# Autodesk Inventor assembly: boil-2
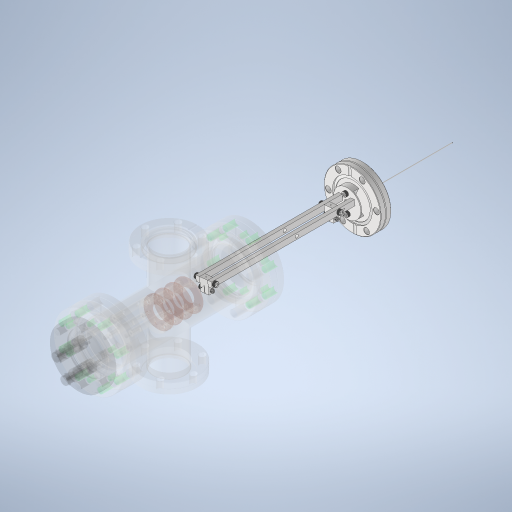
[picture p0: Inventor's stored thumbnail of the model, 512x512]
Saved by Autodesk Inventor 2024 (Build 280153000, 153)
## iProperties
Created: 2023-04-29
Part Number: boil-2
Document SubType Name: Assembly
Designer: Fujitsu
Author: Fujitsu
## Documents named in this file (10)
- C:\Users\Fujitsu\Raad\BaTag\dff275x000\boil-2.iam
- C:\Users\Fujitsu\Raad\BaTag\dff275x000\dff275x000-drilled-2.ipt
- C:\Users\Fujitsu\Raad\BaTag\capillary-2.ipt
- C:\Users\Fujitsu\Raad\BaTag\detector_chamber3\detector_chamber3.iam
- C:\Users\Fujitsu\Raad\BaTag\tab4.ipt
- C:\Users\Fujitsu\Raad\BaTag\rod(6-32).ipt
- C:\Users\Fujitsu\Raad\BaTag\clamp(6-32)-th.ipt
- C:\Users\Fujitsu\Raad\BaTag\ssVScrew(6-32).ipt
- C:\Users\Fujitsu\Raad\BaTag\tee.iam
- C:\Users\Fujitsu\Raad\BaTag\zwj.ipt
## Components (20 placed, 9 different names)
1. dff275x000-drilled-2:1 — Mate:1, Angle:1, Angle:2, Angle:3, Mate:4, Mate:5, Angle:4, Angle:5, Mate:17
2. capillary-2:1 — Mate:1, Angle:1, Mate:2, Mate:3, Mate:6, Mate:11, Mate:15, Mate:16, Mate:18
3. detector_chamber3:1 [sub-assembly] — Angle:2, Mate:2, Mate:3, Mate:20
4. tab4:1 — Angle:3, Mate:4, Mate:5, Mate:6, Mate:7, Mate:8, Mate:9, Mate:10, Insert:1, Insert:2, Insert:3, Insert:4
5. rod(6-32):1 — Mate:9, Mate:10, Angle:4, Mate:12, Mate:13, Mate:14, Insert:5, Insert:8
6. rod(6-32):2 — Mate:7, Mate:8, Angle:5, Insert:9, Insert:10
7. clamp(6-32)-th:1 — Mate:14, Mate:15, Insert:6
8. clamp(6-32)-th:2 — Mate:11, Mate:12, Mate:13, Insert:7
9. ssVScrew(6-32):1 — Insert:8
10. ssVScrew(6-32):2 — Insert:7
11. ssVScrew(6-32):3 — Insert:6
12. ssVScrew(6-32):4 — Insert:5
13. ssVScrew(6-32):5 — Insert:3
14. ssVScrew(6-32):6 — Insert:4
15. ssVScrew(6-32):7 — Insert:2
16. ssVScrew(6-32):8 — Insert:1
17. ssVScrew(6-32):9 — Insert:10
18. ssVScrew(6-32):10 — Insert:9
19. tee:1 [sub-assembly] — Mate:16, Mate:17, Mate:19
20. zwj:1 — Mate:18, Mate:19, Mate:20
## Relationships (35: Mate 20, Insert 10, Angle 5)
- Mate:1: dff275x000-drilled-2:1 ↔ capillary-2:1
- Angle:1 (90 deg): dff275x000-drilled-2:1 ↔ capillary-2:1
- Angle:2 (180 deg): dff275x000-drilled-2:1 ↔ detector_chamber3:1
- Mate:2: capillary-2:1 ↔ detector_chamber3:1
- Mate:3 (15 mm): capillary-2:1 ↔ detector_chamber3:1
- Angle:3 (180 deg): dff275x000-drilled-2:1 ↔ tab4:1
- Mate:4: dff275x000-drilled-2:1 ↔ tab4:1
- Mate:5: dff275x000-drilled-2:1 ↔ tab4:1
- Mate:6: capillary-2:1 ↔ tab4:1
- Mate:7: tab4:1 ↔ rod(6-32):2
- Mate:8: tab4:1 ↔ rod(6-32):2
- Mate:9: tab4:1 ↔ rod(6-32):1
- Mate:10: tab4:1 ↔ rod(6-32):1
- Angle:4 (0 deg): dff275x000-drilled-2:1 ↔ rod(6-32):1
- Angle:5 (0 deg): dff275x000-drilled-2:1 ↔ rod(6-32):2
- Mate:11: capillary-2:1 ↔ clamp(6-32)-th:2
- Mate:12: rod(6-32):1 ↔ clamp(6-32)-th:2
- Mate:13: rod(6-32):1 ↔ clamp(6-32)-th:2
- Mate:14: rod(6-32):1 ↔ clamp(6-32)-th:1
- Mate:15: capillary-2:1 ↔ clamp(6-32)-th:1
- Insert:1: tab4:1 ↔ ssVScrew(6-32):8
- Insert:2: tab4:1 ↔ ssVScrew(6-32):7
- Insert:3: tab4:1 ↔ ssVScrew(6-32):5
- Insert:4: tab4:1 ↔ ssVScrew(6-32):6
- Insert:5: rod(6-32):1 ↔ ssVScrew(6-32):4
- Insert:6: clamp(6-32)-th:1 ↔ ssVScrew(6-32):3
- Insert:7: clamp(6-32)-th:2 ↔ ssVScrew(6-32):2
- Insert:8: rod(6-32):1 ↔ ssVScrew(6-32):1
- Insert:9: rod(6-32):2 ↔ ssVScrew(6-32):10
- Insert:10: rod(6-32):2 ↔ ssVScrew(6-32):9
- Mate:16: capillary-2:1 ↔ tee:1
- Mate:17: dff275x000-drilled-2:1 ↔ tee:1
- Mate:18: capillary-2:1 ↔ zwj:1
- Mate:19: tee:1 ↔ zwj:1
- Mate:20: detector_chamber3:1 ↔ zwj:1
